# Autodesk Inventor assembly: rompe hielos
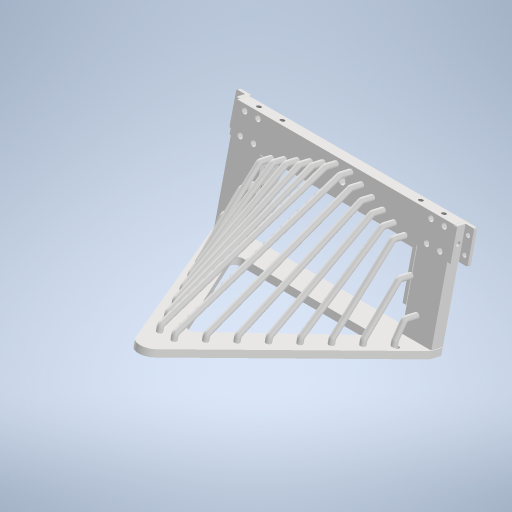
[picture p0: Inventor's stored thumbnail of the model, 512x512]
Saved by Autodesk Inventor 2024.2 (Build 282272000, 272)
## iProperties
Created: 2024-11-02
Part Number: rompe hielos
Document SubType Name: Assembly
Designer: Jimena Brenes
Author: Jimena Brenes
## Documents named in this file (7)
- C:\Users\Jimena Brenes\OneDrive\Escritorio\1-105 rompehielos\rompe hielos.iam
- C:\Users\Jimena Brenes\OneDrive\Escritorio\locomotora\tubos de max.ipt
- C:\Users\Jimena Brenes\OneDrive\Escritorio\PLANOS\pieza 1-19.ipt
- C:\Users\Jimena Brenes\OneDrive\Escritorio\PLANOS\pieza 1-20.ipt
- C:\Users\Jimena Brenes\OneDrive\Escritorio\locomotora\1-18 hudson.ipt
- C:\Users\Jimena Brenes\OneDrive\Escritorio\locomotora en clase\17 nueva.ipt
- C:\Users\Jimena Brenes\OneDrive\Escritorio\locomotora\1-19.ipt
## Components (7 placed, 6 different names)
1. tubos de max:1 — Mate:8, Mate:18
2. pieza 1-19:1 — Mate:11, Mate:12, Mate:13
3. pieza 1-20:1 — Mate:1, Mate:2
4. 1-18 hudson:1 — Mate:1, Mate:2, Mate:3, Mate:4, Mate:5, Mate:8, Mate:9, Mate:10, Mate:11, Mate:12, Mate:13, Mate:14, Mate:15, Mate:16, Mate:17
5. pieza 1-20:2 — Mate:3, Mate:4, Mate:5
6. 17 nueva:1 — Mate:9, Mate:10, Mate:18
7. 1-19:1 — Mate:14, Mate:15, Mate:16, Mate:17
## Relationships (16: Mate 16)
- Mate:1: pieza 1-20:1 ↔ 1-18 hudson:1
- Mate:2: pieza 1-20:1 ↔ 1-18 hudson:1
- Mate:3: 1-18 hudson:1 ↔ pieza 1-20:2
- Mate:4: 1-18 hudson:1 ↔ pieza 1-20:2
- Mate:5: 1-18 hudson:1 ↔ pieza 1-20:2
- Mate:8: tubos de max:1 ↔ 1-18 hudson:1
- Mate:9: 1-18 hudson:1 ↔ 17 nueva:1
- Mate:10: 1-18 hudson:1 ↔ 17 nueva:1
- Mate:11: pieza 1-19:1 ↔ 1-18 hudson:1
- Mate:12: pieza 1-19:1 ↔ 1-18 hudson:1
- Mate:13: pieza 1-19:1 ↔ 1-18 hudson:1
- Mate:14: 1-18 hudson:1 ↔ 1-19:1
- Mate:15: 1-18 hudson:1 ↔ 1-19:1
- Mate:16: 1-18 hudson:1 ↔ 1-19:1
- Mate:17: 1-18 hudson:1 ↔ 1-19:1
- Mate:18: tubos de max:1 ↔ 17 nueva:1
